# Autodesk Inventor assembly: 低速轴
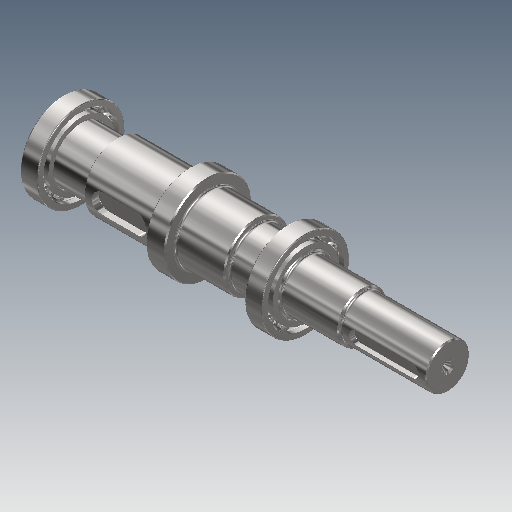
[picture p0: Inventor's stored thumbnail of the model, 512x512]
Saved by Autodesk Inventor 2025 (Build 290162000, 162)
## iProperties
Created: 2025-03-10
Part Number: 低速轴
Document SubType Name: Assembly
Designer: liukan
Author: liukan
## Documents named in this file (3)
- D:\2025春夏那些过往\2025春夏课程文件\机械设计课程设计（甲）\Inventor files\低速轴.iam
- D:\2025春夏那些过往\2025春夏课程文件\机械设计课程设计（甲）\Inventor files\轴3.ipt
- D:\2025春夏那些过往\2025春夏课程文件\机械设计课程设计（甲）\Inventor files\低速轴\设计加速器\轴承1.iam
## Components (3 placed, 2 different names)
1. 轴:1 — 配合:1, 配合:2, 配合:3, 配合:4
2. 轴承:1 [sub-assembly] — 配合:1, 配合:3
3. 轴承:2 [sub-assembly] — 配合:2, 配合:4
## Relationships (4: Mate 4)
- 配合:1 [Mate]: 轴:1 ↔ 轴承:1
- 配合:2 [Mate]: 轴:1 ↔ 轴承:2
- 配合:3 [Mate]: 轴:1 ↔ 轴承:1
- 配合:4 [Mate]: 轴:1 ↔ 轴承:2
